# Autodesk Inventor assembly: Matriz centelladora 15X14
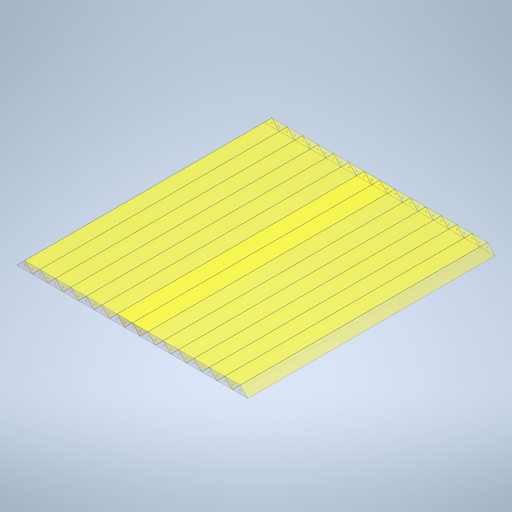
[picture p0: Inventor's stored thumbnail of the model, 512x512]
Saved by Autodesk Inventor 2024.2 (Build 282272000, 272)
## iProperties
Created: 2024-08-22
Part Number: Matriz centelladora 15X14
Document SubType Name: Assembly
Designer: ja.restrepo1
Author: ja.restrepo1
## Documents named in this file (2)
- I:\MICROMECANICA\ALTAS ENERGIAS\Deteccion de Muones\Detectores\Detectores centelladores\Partes Detectores centelladores\PARTES DC\Centelladora DC\SE Matriz centelladora 15X14.iam
- I:\MICROMECANICA\ALTAS ENERGIAS\Deteccion de Muones\Detectores\Detectores centelladores\Partes Detectores centelladores\PARTES DC\Centelladora DC\Centelladora triangular.ipt
## Components (31 placed, 3 different names)
1. Centella origen — Flush:1, Flush:2, Flush:3, Mate:1, Mate:2
2. Centelladora triangular:3
3. Centelladora triangular:4 — Flush:4, Mate:3
4. Centelladora triangular:5
5. Centelladora triangular:6
6. Centelladora triangular:7
7. Centelladora triangular:8
8. Centelladora triangular:9
9. Centelladora triangular:10
10. Centelladora triangular:11
11. Centelladora triangular:12
12. Centelladora triangular:13
13. Centelladora triangular:14
14. Centelladora triangular:15
15. Centelladora triangular:16
16. Centelladora origen 2 — Mate:2, Flush:4, Mate:3
17. Centelladora triangular:17
18. Centelladora triangular:18
19. Centelladora triangular:19
20. Centelladora triangular:20
21. Centelladora triangular:21
22. Centelladora triangular:22
23. Centelladora triangular:23
24. Centelladora triangular:24
25. Centelladora triangular:25
26. Centelladora triangular:26
27. Centelladora triangular:27
28. Centelladora triangular:28
29. Centelladora triangular:29
30. Centelladora triangular:30
31. Centelladora triangular:31
## Component patterns: Matriz 15 (15 elements), Matriz 14 (16 elements)
## Relationships (7: Flush 4, Mate 3)
- Flush:1: Centella origen
- Flush:2: Centella origen
- Flush:3: Centella origen
- Mate:1: Centella origen
- Mate:2: Centella origen ↔ Centelladora origen 2
- Flush:4: Centelladora triangular:4 ↔ Centelladora origen 2
- Mate:3: Centelladora triangular:4 ↔ Centelladora origen 2
